# Autodesk Inventor assembly: BeerMakingShelf
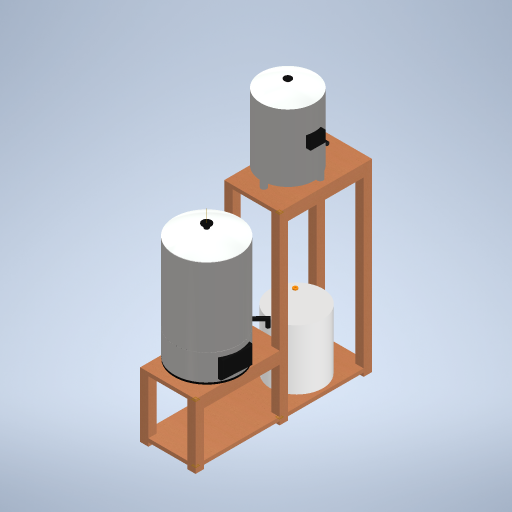
[picture p0: Inventor's stored thumbnail of the model, 512x512]
Saved by Autodesk Inventor 2024 (Build 280153000, 153)
## iProperties
Created: 2025-09-20
Part Number: BeerMakingShelf
Document SubType Name: Assembly
Designer: Emil
Author: Emil
## Documents named in this file (8)
- C:\Users\Emil\OneDrive\Dokument\Projekt-Emil\MachMachine\InventorCad\BeerMakingShelf.iam
- C:\Users\Emil\OneDrive\Dokument\Projekt-Emil\MachMachine\InventorCad\FermentingTun.ipt
- C:\Users\Emil\OneDrive\Dokument\Projekt-Emil\MachMachine\InventorCad\LauteringTun.ipt
- C:\Users\Emil\OneDrive\Dokument\Projekt-Emil\MachMachine\InventorCad\MashMaschine V2.0 modell.ipt
- C:\Users\Emil\OneDrive\Dokument\Projekt-Emil\MachMachine\InventorCad\Shelf.ipt
- C:\Users\Emil\OneDrive\Dokument\Projekt-Emil\MachMachine\InventorCad\shelfBeam.ipt
- C:\Users\Emil\OneDrive\Dokument\Projekt-Emil\MachMachine\InventorCad\selfBeamShort.ipt
- C:\Users\Emil\OneDrive\Dokument\Projekt-Emil\MachMachine\InventorCad\selfBeamLong.ipt
## Components (17 placed, 7 different names)
1. MashMaschine V2.0 modell:1 — Mate:13, Mate:74
2. Shelf:2 — Mate:13, Flush:11, Mate:48, Flush:29, Mate:64, Mate:66, Mate:74, Flush:54
3. LauteringTun:1 — Mate:26, Mate:29, Mate:71
4. Shelf:5 — Flush:24, Mate:42, Mate:43, Flush:26, Mate:45, Mate:46, Mate:47, Flush:31, Flush:32, Flush:33, Mate:52, Mate:53, Flush:34
5. Shelf:6 — Flush:11, Mate:26, Mate:29, Flush:28, Flush:35, Flush:36, Mate:68, Mate:70, Flush:53, Mate:71
6. selfBeamShort:1 — Flush:24, Mate:42, Mate:43, Flush:36
7. selfBeamShort:2 — Flush:26, Mate:45, Mate:46, Flush:28, Flush:35, Flush:52
8. FermentingTun:1 — Mate:47
9. selfBeamShort:4 — Mate:52, Mate:53, Flush:34, Mate:58, Flush:43, Flush:44, Mate:69
10. selfBeamShort:5 — Mate:48, Flush:29, Flush:31, Flush:32, Flush:33, Mate:63, Flush:50, Mate:67
11. Shelf:7 — Mate:58, Flush:43, Flush:44, Mate:59, Flush:45, Flush:46, Mate:60, Mate:61, Flush:47
12. shelfBeam:1 — Mate:59, Flush:45, Flush:46
13. shelfBeam:2 — Mate:60, Mate:61, Flush:47, Mate:65, Flush:51, Flush:54
14. selfBeamLong:1 — Mate:63, Mate:64, Flush:50
15. selfBeamLong:2 — Mate:65, Flush:51, Mate:66
16. selfBeamLong:3 — Mate:69, Mate:70, Flush:52
17. selfBeamLong:4 — Mate:67, Mate:68, Flush:53
## Relationships (46: Mate 25, Flush 21)
- Mate:13: MashMaschine V2.0 modell:1 ↔ Shelf:2
- Flush:11: Shelf:2 ↔ Shelf:6
- Mate:26: LauteringTun:1 ↔ Shelf:6
- Mate:29: LauteringTun:1 ↔ Shelf:6
- Flush:24 (-20 mm): Shelf:5 ↔ selfBeamShort:1
- Mate:42: Shelf:5 ↔ selfBeamShort:1
- Mate:43: Shelf:5 ↔ selfBeamShort:1
- Flush:26 (-20 mm): Shelf:5 ↔ selfBeamShort:2
- Mate:45: Shelf:5 ↔ selfBeamShort:2
- Mate:46: Shelf:5 ↔ selfBeamShort:2
- Flush:28: Shelf:6 ↔ selfBeamShort:2
- Mate:47: Shelf:5 ↔ FermentingTun:1
- Mate:48: Shelf:2 ↔ selfBeamShort:5
- Flush:29: Shelf:2 ↔ selfBeamShort:5
- Flush:31 (-20 mm): Shelf:5 ↔ selfBeamShort:5
- Flush:32: Shelf:5 ↔ selfBeamShort:5
- Flush:33: Shelf:5 ↔ selfBeamShort:5
- Mate:52: Shelf:5 ↔ selfBeamShort:4
- Mate:53: Shelf:5 ↔ selfBeamShort:4
- Flush:34 (20 mm): Shelf:5 ↔ selfBeamShort:4
- Flush:35: Shelf:6 ↔ selfBeamShort:2
- Flush:36: Shelf:6 ↔ selfBeamShort:1
- Mate:58: selfBeamShort:4 ↔ Shelf:7
- Flush:43: selfBeamShort:4 ↔ Shelf:7
- Flush:44 (20 mm): selfBeamShort:4 ↔ Shelf:7
- Mate:59: Shelf:7 ↔ shelfBeam:1
- Flush:45: Shelf:7 ↔ shelfBeam:1
- Flush:46 (-20 mm): Shelf:7 ↔ shelfBeam:1
- Mate:60: Shelf:7 ↔ shelfBeam:2
- Mate:61: Shelf:7 ↔ shelfBeam:2
- Flush:47 (-20 mm): Shelf:7 ↔ shelfBeam:2
- Mate:63: selfBeamShort:5 ↔ selfBeamLong:1
- Mate:64: Shelf:2 ↔ selfBeamLong:1
- Flush:50: selfBeamShort:5 ↔ selfBeamLong:1
- Mate:65: shelfBeam:2 ↔ selfBeamLong:2
- Flush:51: shelfBeam:2 ↔ selfBeamLong:2
- Mate:66: Shelf:2 ↔ selfBeamLong:2
- Mate:67: selfBeamShort:5 ↔ selfBeamLong:4
- Mate:68: Shelf:6 ↔ selfBeamLong:4
- Mate:69: selfBeamShort:4 ↔ selfBeamLong:3
- Mate:70: Shelf:6 ↔ selfBeamLong:3
- Flush:52: selfBeamShort:2 ↔ selfBeamLong:3
- Flush:53: Shelf:6 ↔ selfBeamLong:4
- Mate:71: LauteringTun:1 ↔ Shelf:6
- Mate:74: MashMaschine V2.0 modell:1 ↔ Shelf:2
- Flush:54: Shelf:2 ↔ shelfBeam:2
